# Autodesk Inventor assembly: MG_996R
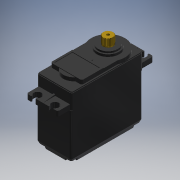
[picture p0: Inventor's stored thumbnail of the model, 180x180]
Saved by Autodesk Inventor 2019 (Build 230136000, 136)
## iProperties
Created: 2016-09-26
Part Number: MG_996R
Document SubType Name: Assembly
Designer: Julian
Author: Julian
## Documents named in this file (6)
- E:\Escritorio\Temporal\Documentos\Robótica I\Robótica I - Proyecto Cuadrúpedo\Servo MG996R\Servo MG996R - Ensamble - Sin Flor.iam
- E:\Escritorio\Temporal\Documentos\Robótica I\Robótica I - Proyecto Cuadrúpedo\Servo MG996R\TowerPro SG5010 - Base.ipt
- E:\Escritorio\Temporal\Documentos\Robótica I\Robótica I - Proyecto Cuadrúpedo\Servo MG996R\TowerPro SG5010 - Medio.ipt
- E:\Escritorio\Temporal\Documentos\Robótica I\Robótica I - Proyecto Cuadrúpedo\Servo MG996R\TowerPro SG5010 - Tapa Superior.ipt
- E:\Escritorio\Temporal\Documentos\Robótica I\Robótica I - Proyecto Cuadrúpedo\Servo MG996R\TowerPro SG5010 - Eje.ipt
- E:\Escritorio\Temporal\Documentos\Robótica I\Robótica I - Proyecto Cuadrúpedo\Servo MG996R\TowerPro SG5010 - Acople Circular.ipt
## Components (5 placed, 5 different names)
1. TowerPro SG5010 - Tapa Superior:1 — Rígido:2, De rotación:1
2. TowerPro SG5010 - Medio:1 — Rígido:1, Rígido:2
3. TowerPro SG5010 - Base:1 — Rígido:1
4. TowerPro SG5010 - Eje:1 — De rotación:1, De rotación:2
5. TowerPro SG5010 - Acople Circular:1 — De rotación:2
## Relationships (4: WeldJoint 2, RevoluteJoint 2)
- Rígido:1 [WeldJoint]: TowerPro SG5010 - Medio:1 ↔ TowerPro SG5010 - Base:1
- Rígido:2 [WeldJoint]: TowerPro SG5010 - Tapa Superior:1 ↔ TowerPro SG5010 - Medio:1
- De rotación:1 [RevoluteJoint]: TowerPro SG5010 - Tapa Superior:1 ↔ TowerPro SG5010 - Eje:1
- De rotación:2 [RevoluteJoint]: TowerPro SG5010 - Eje:1 ↔ TowerPro SG5010 - Acople Circular:1
